# Autodesk Inventor assembly: Planta
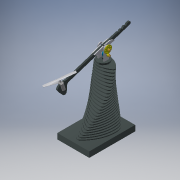
[picture p0: Inventor's stored thumbnail of the model, 180x180]
Saved by Autodesk Inventor 2016 (Build 200138000, 138)
## iProperties
Created: 2016-09-20
Part Number: Planta
Material: Genérico
Document SubType Name: Assembly
Designer: i95sa
Author: i95sa
## Documents named in this file (41)
- C:\Users\i95sa\Documents\Universidad\semestre X\Técnicas de control\proyecto\modelo3D02Laser\Planta.iam
- C:\Users\i95sa\Documents\Universidad\semestre X\Técnicas de control\proyecto\modelo3D02Laser\levas\leva00.ipt
- C:\Users\i95sa\Documents\Universidad\semestre X\Técnicas de control\proyecto\modelo3D02Laser\entreCapa8mm.ipt
- C:\Users\i95sa\Documents\Universidad\semestre X\Técnicas de control\proyecto\modelo3D02Laser\levas\leva00 - copia.ipt
- C:\Users\i95sa\Documents\Universidad\semestre X\Técnicas de control\proyecto\modelo3D02Laser\levas\leva00 - copia (2).ipt
- C:\Users\i95sa\Documents\Universidad\semestre X\Técnicas de control\proyecto\modelo3D02Laser\levas\leva00 - copia (3).ipt
- C:\Users\i95sa\Documents\Universidad\semestre X\Técnicas de control\proyecto\modelo3D02Laser\levas\leva00 - copia (4).ipt
- C:\Users\i95sa\Documents\Universidad\semestre X\Técnicas de control\proyecto\modelo3D02Laser\levas\leva00 - copia (5).ipt
- C:\Users\i95sa\Documents\Universidad\semestre X\Técnicas de control\proyecto\modelo3D02Laser\levas\leva00 - copia (6).ipt
- C:\Users\i95sa\Documents\Universidad\semestre X\Técnicas de control\proyecto\modelo3D02Laser\levas\leva00 - copia (7).ipt
- C:\Users\i95sa\Documents\Universidad\semestre X\Técnicas de control\proyecto\modelo3D02Laser\levas\leva00 - copia (8).ipt
- C:\Users\i95sa\Documents\Universidad\semestre X\Técnicas de control\proyecto\modelo3D02Laser\levas\leva00 - copia (9).ipt
- C:\Users\i95sa\Documents\Universidad\semestre X\Técnicas de control\proyecto\modelo3D02Laser\levas\leva00 - copia (10).ipt
- C:\Users\i95sa\Documents\Universidad\semestre X\Técnicas de control\proyecto\modelo3D02Laser\levas\leva00 - copia (11).ipt
- C:\Users\i95sa\Documents\Universidad\semestre X\Técnicas de control\proyecto\modelo3D02Laser\levas\leva00 - copia (12).ipt
- C:\Users\i95sa\Documents\Universidad\semestre X\Técnicas de control\proyecto\modelo3D02Laser\levas\leva00 - copia (13).ipt
- C:\Users\i95sa\Documents\Universidad\semestre X\Técnicas de control\proyecto\modelo3D02Laser\levas\leva00 - copia (14).ipt
- C:\Users\i95sa\Documents\Universidad\semestre X\Técnicas de control\proyecto\modelo3D02Laser\levas\leva00 - copia (15).ipt
- C:\Users\i95sa\Documents\Universidad\semestre X\Técnicas de control\proyecto\modelo3D02Laser\levas\leva00 - copia (16).ipt
- C:\Users\i95sa\Documents\Universidad\semestre X\Técnicas de control\proyecto\modelo3D02Laser\levas\leva00 - copia (17).ipt
- C:\Users\i95sa\Documents\Universidad\semestre X\Técnicas de control\proyecto\modelo3D02Laser\levas\leva00 - copia (18).ipt
- C:\Users\i95sa\Documents\Universidad\semestre X\Técnicas de control\proyecto\modelo3D02Laser\levas\leva00 - copia (19).ipt
- C:\Users\i95sa\Documents\Universidad\semestre X\Técnicas de control\proyecto\modelo3D02Laser\levas\leva00 - copia (20).ipt
- C:\Users\i95sa\Documents\Universidad\semestre X\Técnicas de control\proyecto\modelo3D02Laser\levas\leva00 - copia (21).ipt
- C:\Users\i95sa\Documents\Universidad\semestre X\Técnicas de control\proyecto\modelo3D02Laser\levas\leva00 - copia (22).ipt
- C:\Users\i95sa\Documents\Universidad\semestre X\Técnicas de control\proyecto\modelo3D02Laser\levas\leva00 - copia (23).ipt
- C:\Users\i95sa\Documents\Universidad\semestre X\Técnicas de control\proyecto\modelo3D02Laser\columna01.ipt
- C:\Users\i95sa\Documents\Universidad\semestre X\Técnicas de control\proyecto\modelo3D02Laser\columna02.ipt
- C:\Users\i95sa\Documents\Universidad\semestre X\Técnicas de control\proyecto\modelo3D02Laser\rodamiento.ipt
- C:\Users\i95sa\Documents\Universidad\semestre X\Técnicas de control\proyecto\modelo3D02Laser\potenciometro.ipt
- C:\Users\i95sa\Documents\Universidad\semestre X\Técnicas de control\proyecto\modelo3D02Laser\eje.ipt
- C:\Users\i95sa\Documents\Universidad\semestre X\Técnicas de control\proyecto\modelo3D02Laser\engraneGrande.ipt
- C:\Users\i95sa\Documents\Universidad\semestre X\Técnicas de control\proyecto\modelo3D02Laser\engranePeq.ipt
- C:\Users\i95sa\Documents\Universidad\semestre X\Técnicas de control\proyecto\modelo3D02Laser\base.ipt
- C:\Users\i95sa\Documents\Universidad\semestre X\Técnicas de control\proyecto\modelo3D02Laser\base1.ipt
- C:\Users\i95sa\Documents\Universidad\semestre X\Técnicas de control\proyecto\modelo3D02Laser\base2.ipt
- C:\Users\i95sa\Documents\Universidad\semestre X\Técnicas de control\proyecto\modelo3D02Laser\base3.ipt
- C:\Users\i95sa\Documents\Universidad\semestre X\Técnicas de control\proyecto\modelo3D02Laser\balancin.ipt
- C:\Users\i95sa\Documents\Universidad\semestre X\Técnicas de control\proyecto\modelo3D02Laser\balancinRefuerzos.ipt
- C:\Users\i95sa\Documents\Universidad\semestre X\Técnicas de control\proyecto\modelo3D02Laser\MotorCesar.ipt
- C:\Users\i95sa\Documents\Universidad\semestre X\Técnicas de control\proyecto\modelo3D02Laser\helice.ipt
## Components (67 placed, 40 different names)
1. leva00:1 — Insertar:1, Nivelación:1, Coincidencia:1, Coincidencia:2, Nivelación:2, Coincidencia:3, Coincidencia:4, Insertar:54
2. entreCapa8mm:1 — Insertar:1, Insertar:2
3. leva00 - copia:1 — Insertar:2, Insertar:3
4. leva00 - copia (2):1 — Insertar:4, Insertar:5
5. leva00 - copia (3):1 — Insertar:6, Insertar:7
6. leva00 - copia (4):1 — Insertar:8, Insertar:47
7. leva00 - copia (5):1 — Insertar:9, Insertar:46
8. leva00 - copia (6):1 — Insertar:10, Insertar:45
9. leva00 - copia (7):1 — Insertar:11, Insertar:44
10. leva00 - copia (8):1 — Insertar:12, Insertar:43
11. leva00 - copia (9):1 — Insertar:13, Insertar:42
12. leva00 - copia (10):1 — Insertar:14, Insertar:41
13. leva00 - copia (11):1 — Insertar:15, Insertar:40
14. leva00 - copia (12):1 — Insertar:16, Insertar:39
15. leva00 - copia (13):1 — Insertar:17, Insertar:38
16. leva00 - copia (14):1 — Insertar:18, Insertar:37
17. leva00 - copia (15):1 — Insertar:19, Insertar:36
18. leva00 - copia (16):1 — Insertar:20, Insertar:35
19. leva00 - copia (17):1 — Insertar:21, Insertar:34
20. leva00 - copia (18):1 — Insertar:22, Insertar:33
21. leva00 - copia (19):1 — Insertar:23, Insertar:32
22. leva00 - copia (20):1 — Insertar:24, Insertar:31
23. leva00 - copia (21):1 — Insertar:25, Insertar:30
24. leva00 - copia (22):1 — Insertar:26, Insertar:29
25. leva00 - copia (23):1 — Insertar:27, Insertar:28
26. entreCapa8mm:2 — Insertar:3, Insertar:4
27. entreCapa8mm:3 — Insertar:5, Insertar:6
28. entreCapa8mm:4 — Insertar:7, Insertar:8
29. entreCapa8mm:5 — Insertar:9, Insertar:45
30. entreCapa8mm:6 — Insertar:10, Insertar:44
31. entreCapa8mm:7 — Insertar:11, Insertar:43
32. entreCapa8mm:8 — Insertar:12, Insertar:42
33. entreCapa8mm:9 — Insertar:13, Insertar:41
34. entreCapa8mm:10 — Insertar:14, Insertar:40
35. entreCapa8mm:11 — Insertar:15, Insertar:39
36. entreCapa8mm:12 — Insertar:16, Insertar:38
37. entreCapa8mm:13 — Insertar:17, Insertar:37
38. entreCapa8mm:14 — Insertar:18, Insertar:36
39. entreCapa8mm:15 — Insertar:19, Insertar:35
40. entreCapa8mm:16 — Insertar:20, Insertar:34
41. entreCapa8mm:17 — Insertar:21, Insertar:33
42. entreCapa8mm:18 — Insertar:22, Insertar:32
43. entreCapa8mm:19 — Insertar:23, Insertar:31
44. entreCapa8mm:20 — Insertar:24, Insertar:30
45. entreCapa8mm:21 — Insertar:25, Insertar:29
46. entreCapa8mm:22 — Insertar:26, Insertar:28
47. entreCapa8mm:23 — Insertar:27
48. entreCapa8mm:24 — Insertar:46, Insertar:47
49. columna01:1 — Nivelación:1, Coincidencia:1, Coincidencia:2, Insertar:48, Insertar:50, Ángulo:1, Insertar:53, Ángulo:2
50. rodamiento:1 — Insertar:48
51. rodamiento:2 — Insertar:49, Insertar:51
52. potenciometro:1 — Insertar:50, Ángulo:1, Insertar:52
53. eje:1 — Insertar:51, Insertar:55, Coincidencia:12, Rotación:2
54. engraneGrande:1 — Insertar:53, Rotación:1, Rotación:2
55. engranePeq:1 — Insertar:52, Rotación:1
56. base:1 — Ángulo:2, Insertar:54, Coincidencia:5, Coincidencia:6, Coincidencia:7, Coincidencia:8, Nivelación:3, Nivelación:4, Nivelación:5, Nivelación:6, Nivelación:7, Nivelación:8
57. base1:1 — Coincidencia:6, Nivelación:5, Nivelación:6, Coincidencia:9, Nivelación:10
58. base2:1 — Coincidencia:8, Nivelación:8, Coincidencia:10, Nivelación:9, Coincidencia:11
59. base1:2 — Coincidencia:5, Nivelación:3, Nivelación:4, Coincidencia:10
60. base2:2 — Coincidencia:7, Nivelación:7, Coincidencia:9
61. base3:1 — Nivelación:9, Nivelación:10, Coincidencia:11
62. balancin:1 — Insertar:55, Coincidencia:12, Insertar:56, Nivelación:11, Insertar:57, Nivelación:12, Coincidencia:13, Coincidencia:14, Coincidencia:15
63. balancinRefuerzos:1 — Insertar:56, Nivelación:11
64. balancinRefuerzos:2 — Insertar:57, Nivelación:12
65. MotorCesar:1 — Coincidencia:13, Coincidencia:14, Coincidencia:15, Insertar:58
66. helice:1 — Insertar:58
67. columna02:1 — Nivelación:2, Coincidencia:3, Coincidencia:4, Insertar:49
## Relationships (89: Insert 58, Mate 15, Flush 12, Angle 2, RelateRotation 2)
- Insertar:1: leva00:1 ↔ entreCapa8mm:1
- Insertar:2: entreCapa8mm:1 ↔ leva00 - copia:1
- Insertar:3: leva00 - copia:1 ↔ entreCapa8mm:2
- Insertar:4: leva00 - copia (2):1 ↔ entreCapa8mm:2
- Insertar:5: leva00 - copia (2):1 ↔ entreCapa8mm:3
- Insertar:6: leva00 - copia (3):1 ↔ entreCapa8mm:3
- Insertar:7: leva00 - copia (3):1 ↔ entreCapa8mm:4
- Insertar:8: leva00 - copia (4):1 ↔ entreCapa8mm:4
- Insertar:9: leva00 - copia (5):1 ↔ entreCapa8mm:5
- Insertar:10: leva00 - copia (6):1 ↔ entreCapa8mm:6
- Insertar:11: leva00 - copia (7):1 ↔ entreCapa8mm:7
- Insertar:12: leva00 - copia (8):1 ↔ entreCapa8mm:8
- Insertar:13: leva00 - copia (9):1 ↔ entreCapa8mm:9
- Insertar:14: leva00 - copia (10):1 ↔ entreCapa8mm:10
- Insertar:15: leva00 - copia (11):1 ↔ entreCapa8mm:11
- Insertar:16: leva00 - copia (12):1 ↔ entreCapa8mm:12
- Insertar:17: leva00 - copia (13):1 ↔ entreCapa8mm:13
- Insertar:18: leva00 - copia (14):1 ↔ entreCapa8mm:14
- Insertar:19: leva00 - copia (15):1 ↔ entreCapa8mm:15
- Insertar:20: leva00 - copia (16):1 ↔ entreCapa8mm:16
- Insertar:21: leva00 - copia (17):1 ↔ entreCapa8mm:17
- Insertar:22: leva00 - copia (18):1 ↔ entreCapa8mm:18
- Insertar:23: leva00 - copia (19):1 ↔ entreCapa8mm:19
- Insertar:24: leva00 - copia (20):1 ↔ entreCapa8mm:20
- Insertar:25: leva00 - copia (21):1 ↔ entreCapa8mm:21
- Insertar:26: leva00 - copia (22):1 ↔ entreCapa8mm:22
- Insertar:27: leva00 - copia (23):1 ↔ entreCapa8mm:23
- Insertar:28: leva00 - copia (23):1 ↔ entreCapa8mm:22
- Insertar:29: leva00 - copia (22):1 ↔ entreCapa8mm:21
- Insertar:30: leva00 - copia (21):1 ↔ entreCapa8mm:20
- Insertar:31: leva00 - copia (20):1 ↔ entreCapa8mm:19
- Insertar:32: leva00 - copia (19):1 ↔ entreCapa8mm:18
- Insertar:33: leva00 - copia (18):1 ↔ entreCapa8mm:17
- Insertar:34: leva00 - copia (17):1 ↔ entreCapa8mm:16
- Insertar:35: leva00 - copia (16):1 ↔ entreCapa8mm:15
- Insertar:36: leva00 - copia (15):1 ↔ entreCapa8mm:14
- Insertar:37: leva00 - copia (14):1 ↔ entreCapa8mm:13
- Insertar:38: leva00 - copia (13):1 ↔ entreCapa8mm:12
- Insertar:39: leva00 - copia (12):1 ↔ entreCapa8mm:11
- Insertar:40: leva00 - copia (11):1 ↔ entreCapa8mm:10
- Insertar:41: leva00 - copia (10):1 ↔ entreCapa8mm:9
- Insertar:42: leva00 - copia (9):1 ↔ entreCapa8mm:8
- Insertar:43: leva00 - copia (8):1 ↔ entreCapa8mm:7
- Insertar:44: leva00 - copia (7):1 ↔ entreCapa8mm:6
- Insertar:45: leva00 - copia (6):1 ↔ entreCapa8mm:5
- Insertar:46: leva00 - copia (5):1 ↔ entreCapa8mm:24
- Insertar:47: leva00 - copia (4):1 ↔ entreCapa8mm:24
- Nivelación:1 [Flush]: leva00:1 ↔ columna01:1
- Coincidencia:1 [Mate]: leva00:1 ↔ columna01:1
- Coincidencia:2 [Mate]: leva00:1 ↔ columna01:1
- Nivelación:2 [Flush]: leva00:1 ↔ columna02:1
- Coincidencia:3 [Mate]: leva00:1 ↔ columna02:1
- Coincidencia:4 [Mate]: leva00:1 ↔ columna02:1
- Insertar:48: columna01:1 ↔ rodamiento:1
- Insertar:49: rodamiento:2 ↔ columna02:1
- Insertar:50 (2 mm): columna01:1 ↔ potenciometro:1
- Ángulo:1 [Angle] (0 deg): columna01:1 ↔ potenciometro:1
- Insertar:51 (-5 mm): rodamiento:2 ↔ eje:1
- Insertar:52: potenciometro:1 ↔ engranePeq:1
- Insertar:53 (6 mm): columna01:1 ↔ engraneGrande:1
- Rotación:1 [RelateRotation] (3 ul): engraneGrande:1 ↔ engranePeq:1
- Ángulo:2 [Angle] (180 deg): columna01:1 ↔ base:1
- Insertar:54: leva00:1 ↔ base:1
- Coincidencia:5 [Mate]: base:1 ↔ base1:2
- Coincidencia:6 [Mate]: base:1 ↔ base1:1
- Coincidencia:7 [Mate]: base:1 ↔ base2:2
- Coincidencia:8 [Mate]: base:1 ↔ base2:1
- Nivelación:3 [Flush]: base:1 ↔ base1:2
- Nivelación:4 [Flush]: base:1 ↔ base1:2
- Nivelación:5 [Flush]: base:1 ↔ base1:1
- Nivelación:6 [Flush]: base:1 ↔ base1:1
- Nivelación:7 [Flush]: base:1 ↔ base2:2
- Nivelación:8 [Flush]: base:1 ↔ base2:1
- Coincidencia:9 [Mate]: base1:1 ↔ base2:2
- Coincidencia:10 [Mate]: base2:1 ↔ base1:2
- Nivelación:9 [Flush]: base2:1 ↔ base3:1
- Nivelación:10 [Flush]: base1:1 ↔ base3:1
- Coincidencia:11 [Mate]: base2:1 ↔ base3:1
- Insertar:55 (6 mm): eje:1 ↔ balancin:1
- Coincidencia:12 [Mate]: eje:1 ↔ balancin:1
- Rotación:2 [RelateRotation] (1 ul): eje:1 ↔ engraneGrande:1
- Insertar:56: balancin:1 ↔ balancinRefuerzos:1
- Nivelación:11 [Flush]: balancin:1 ↔ balancinRefuerzos:1
- Insertar:57: balancin:1 ↔ balancinRefuerzos:2
- Nivelación:12 [Flush]: balancin:1 ↔ balancinRefuerzos:2
- Coincidencia:13 [Mate]: balancin:1 ↔ MotorCesar:1
- Coincidencia:14 [Mate]: balancin:1 ↔ MotorCesar:1
- Coincidencia:15 [Mate] (-4 mm): balancin:1 ↔ MotorCesar:1
- Insertar:58 (2 mm): MotorCesar:1 ↔ helice:1
